# Autodesk Inventor assembly: Rover_komplett
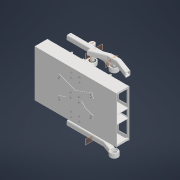
[picture p0: Inventor's stored thumbnail of the model, 180x180]
Saved by Autodesk Inventor 2021 (Build 250183000, 183)
## iProperties
Created: 2021-03-06
Part Number: Rover_komplett
Document SubType Name: Assembly
Designer: Ctroi
Author: Ctroi
## Documents named in this file (25)
- G:\Roverprojekt\Github Projekt\Rover\Rover_komplett.iam
- G:\Roverprojekt\Github Projekt\Rover\Grundplatte_vorne.ipt
- G:\Roverprojekt\Github Projekt\Rover\Grundplatte_hinten.ipt
- G:\Roverprojekt\Github Projekt\Rover\Obenplatte_vorne.ipt
- C:\Users\Ctroi\Documents\Inventor\Content Center Files\R2021\de-DE\ISO 7089\ISO 7089 - 3 - 140 HV(1).ipt
- C:\Users\Ctroi\Documents\Inventor\Content Center Files\R2021\de-DE\BS 4168(1)\BS 4168 - M3 x 10(1).ipt
- C:\Users\Ctroi\Documents\Inventor\Content Center Files\R2021\de-DE\ANSI B18.16.3M(2)\ANSI B18.16.3M - Property Class 5 and 10 - Metric M3 x 0.5 Metallisch.ipt
- G:\Roverprojekt\Github Projekt\Rover\Kreuz_Halterung.ipt
- C:\Users\Ctroi\Documents\Inventor\Content Center Files\R2021\de-DE\BS 4168(1)\BS 4168 - M3 x 8(1).ipt
- G:\Roverprojekt\Github Projekt\Rover\Obenplatte_hinten.ipt
- G:\Roverprojekt\Github Projekt\Rover\Halterung_Differential_3.ipt
- C:\Users\Ctroi\Documents\Inventor\Content Center Files\R2021\de-DE\BS 4168(1)\BS 4168 - M3 x 12(1).ipt
- G:\Roverprojekt\Github Projekt\Rover\Halterung_Differential.ipt
- G:\Roverprojekt\Github Projekt\Rover\Halterung_Differential_2.ipt
- G:\Roverprojekt\Github Projekt\Rover\Kugellager.ipt
- G:\Roverprojekt\Github Projekt\Rover\Halterung_Differential_Mitte.ipt
- G:\Roverprojekt\Github Projekt\Rover\Kugellager_klein.ipt
- G:\Roverprojekt\Github Projekt\Rover\Welle_Kugellager_Mitte.ipt
- G:\Roverprojekt\Github Projekt\Rover\Kegelrad.ipt
- G:\Roverprojekt\Github Projekt\Rover\Verbindung_Rocker_Body.ipt
- C:\Users\Ctroi\Documents\Inventor\Content Center Files\R2021\de-DE\BS 4168(1)\BS 4168 - M3 x 16(1).ipt
- G:\Roverprojekt\Github Projekt\Rover\Rocker_hinten.ipt
- G:\Roverprojekt\Github Projekt\Rover\Rocker_hinten_rechts.ipt
- G:\Roverprojekt\Github Projekt\Rover\Boogie_Stange.ipt
- G:\Roverprojekt\Github Projekt\Rover\Bogie.ipt
## Components (165 placed, 23 different names)
1. Fahrwerk_rocker_hinten:1 — Passend:196, Passend:197, Winkel:8, Passend:200, Passend:201, Passend:202, Passend:203
2. Fahrwerk_rocker_hinten:2 — Passend:198, Passend:199, Winkel:9
3. Kugellager:6 — Passend:200, Passend:201, Einfügen:72
4. Kugellager:7 — Passend:202, Passend:203
5. Boogie_Stange:1 — Einfügen:72, Passend:204, Passend:205, Winkel:10
6. Fahrwerk_bogie:1 — Passend:204, Passend:205, Winkel:10
7. ISO 7089 3:17 — Passend:46, Passend:47, Einfügen:17
8. BS 4168 : Teil 1 Innensechskantschraube - Metrisch M3 x 8:1 — Einfügen:17
9. ISO 7089 3:18 — Passend:48, Passend:49, Einfügen:18
10. Sechskantmutter mit Sicherungselement - Stahl Metrisch Property Class 5 and 10 - Metric M3 x 0.5 Metallisch:9 — Einfügen:18
11. ISO 7089 3:19 — Passend:50, Passend:51, Einfügen:19
12. BS 4168 : Teil 1 Innensechskantschraube - Metrisch M3 x 8:2 — Einfügen:19
13. ISO 7089 3:20 — Passend:52, Passend:53, Einfügen:20
14. Sechskantmutter mit Sicherungselement - Stahl Metrisch Property Class 5 and 10 - Metric M3 x 0.5 Metallisch:10 — Einfügen:20
15. ISO 7089 3:21 — Passend:54, Passend:55, Einfügen:21
16. BS 4168 : Teil 1 Innensechskantschraube - Metrisch M3 x 8:3 — Einfügen:21
17. ISO 7089 3:22 — Passend:56, Passend:57, Einfügen:22
18. Sechskantmutter mit Sicherungselement - Stahl Metrisch Property Class 5 and 10 - Metric M3 x 0.5 Metallisch:11 — Einfügen:22
19. ISO 7089 3:23 — Passend:58, Passend:59, Einfügen:23
20. BS 4168 : Teil 1 Innensechskantschraube - Metrisch M3 x 8:4 — Einfügen:23
21. ISO 7089 3:24 — Passend:60, Passend:61, Einfügen:24
22. Sechskantmutter mit Sicherungselement - Stahl Metrisch Property Class 5 and 10 - Metric M3 x 0.5 Metallisch:12 — Einfügen:24
23. ISO 7089 3:25 — Passend:62, Passend:63, Einfügen:25
24. BS 4168 : Teil 1 Innensechskantschraube - Metrisch M3 x 8:5 — Einfügen:25
25. ISO 7089 3:26 — Passend:64, Passend:65, Einfügen:26
26. Sechskantmutter mit Sicherungselement - Stahl Metrisch Property Class 5 and 10 - Metric M3 x 0.5 Metallisch:13 — Einfügen:26
27. ISO 7089 3:27 — Passend:66, Passend:67, Einfügen:27
28. BS 4168 : Teil 1 Innensechskantschraube - Metrisch M3 x 10:9 — Einfügen:27
29. ISO 7089 3:28 — Passend:68, Passend:69, Einfügen:28
30. Sechskantmutter mit Sicherungselement - Stahl Metrisch Property Class 5 and 10 - Metric M3 x 0.5 Metallisch:14 — Einfügen:28
31. ISO 7089 3:29 — Passend:70, Passend:71, Einfügen:29
32. BS 4168 : Teil 1 Innensechskantschraube - Metrisch M3 x 10:10 — Einfügen:29
33. ISO 7089 3:30 — Passend:72, Passend:73, Einfügen:30
34. Sechskantmutter mit Sicherungselement - Stahl Metrisch Property Class 5 and 10 - Metric M3 x 0.5 Metallisch:15 — Einfügen:30
35. ISO 7089 3:31 — Passend:74, Passend:75, Einfügen:31
36. BS 4168 : Teil 1 Innensechskantschraube - Metrisch M3 x 10:11 — Einfügen:31
37. ISO 7089 3:32 — Passend:76, Passend:77, Einfügen:32
38. Sechskantmutter mit Sicherungselement - Stahl Metrisch Property Class 5 and 10 - Metric M3 x 0.5 Metallisch:16 — Einfügen:32
39. ISO 7089 3:33 — Passend:78, Passend:79, Einfügen:33
40. BS 4168 : Teil 1 Innensechskantschraube - Metrisch M3 x 10:12 — Einfügen:33
41. ISO 7089 3:34 — Passend:80, Passend:81, Einfügen:34
42. Sechskantmutter mit Sicherungselement - Stahl Metrisch Property Class 5 and 10 - Metric M3 x 0.5 Metallisch:17 — Einfügen:34
43. ISO 7089 3:35 — Passend:82, Passend:83, Einfügen:35
44. BS 4168 : Teil 1 Innensechskantschraube - Metrisch M3 x 10:13 — Einfügen:35
45. ISO 7089 3:36 — Passend:84, Passend:85, Einfügen:36
46. Sechskantmutter mit Sicherungselement - Stahl Metrisch Property Class 5 and 10 - Metric M3 x 0.5 Metallisch:18 — Einfügen:36
47. ISO 7089 3:37 — Passend:86, Passend:87, Einfügen:37
48. BS 4168 : Teil 1 Innensechskantschraube - Metrisch M3 x 10:14 — Einfügen:37
49. ISO 7089 3:38 — Passend:88, Passend:89, Einfügen:38
50. Sechskantmutter mit Sicherungselement - Stahl Metrisch Property Class 5 and 10 - Metric M3 x 0.5 Metallisch:19 — Einfügen:38
51. ISO 7089 3:39 — Passend:90, Passend:91, Einfügen:39
52. BS 4168 : Teil 1 Innensechskantschraube - Metrisch M3 x 10:15 — Einfügen:39
53. ISO 7089 3:40 — Passend:92, Passend:93, Einfügen:40
54. Sechskantmutter mit Sicherungselement - Stahl Metrisch Property Class 5 and 10 - Metric M3 x 0.5 Metallisch:20 — Einfügen:40
55. ISO 7089 3:1 — Passend:11, Passend:12, Einfügen:1
56. BS 4168 : Teil 1 Innensechskantschraube - Metrisch M3 x 10:1 — Einfügen:1
57. ISO 7089 3:2 — Passend:13, Passend:14, Einfügen:2
58. Sechskantmutter mit Sicherungselement - Stahl Metrisch Property Class 5 and 10 - Metric M3 x 0.5 Metallisch:1 — Einfügen:2
59. ISO 7089 3:3 — Passend:15, Passend:16, Einfügen:3
60. BS 4168 : Teil 1 Innensechskantschraube - Metrisch M3 x 10:2 — Einfügen:3
61. ISO 7089 3:4 — Passend:17, Passend:18, Einfügen:4
62. Sechskantmutter mit Sicherungselement - Stahl Metrisch Property Class 5 and 10 - Metric M3 x 0.5 Metallisch:2 — Einfügen:4
63. ISO 7089 3:5 — Passend:19, Passend:20, Einfügen:5
64. BS 4168 : Teil 1 Innensechskantschraube - Metrisch M3 x 10:3 — Einfügen:5
65. ISO 7089 3:6 — Passend:21, Passend:22, Einfügen:6
66. Sechskantmutter mit Sicherungselement - Stahl Metrisch Property Class 5 and 10 - Metric M3 x 0.5 Metallisch:3 — Einfügen:6
67. ISO 7089 3:7 — Passend:23, Passend:24, Einfügen:7
68. BS 4168 : Teil 1 Innensechskantschraube - Metrisch M3 x 10:4 — Einfügen:7
69. ISO 7089 3:8 — Passend:25, Passend:26, Einfügen:8
70. Sechskantmutter mit Sicherungselement - Stahl Metrisch Property Class 5 and 10 - Metric M3 x 0.5 Metallisch:4 — Einfügen:8
71. ISO 7089 3:9 — Passend:27, Passend:28, Einfügen:9
72. BS 4168 : Teil 1 Innensechskantschraube - Metrisch M3 x 10:5 — Einfügen:9
73. ISO 7089 3:10 — Passend:29, Passend:30, Einfügen:10
74. Sechskantmutter mit Sicherungselement - Stahl Metrisch Property Class 5 and 10 - Metric M3 x 0.5 Metallisch:5 — Einfügen:10
75. ISO 7089 3:11 — Passend:31, Passend:32, Einfügen:11
76. BS 4168 : Teil 1 Innensechskantschraube - Metrisch M3 x 10:6 — Einfügen:11
77. ISO 7089 3:12 — Passend:33, Passend:34, Einfügen:12
78. Sechskantmutter mit Sicherungselement - Stahl Metrisch Property Class 5 and 10 - Metric M3 x 0.5 Metallisch:6 — Einfügen:12
79. ISO 7089 3:13 — Passend:35, Passend:36, Einfügen:13
80. BS 4168 : Teil 1 Innensechskantschraube - Metrisch M3 x 10:7 — Einfügen:13
81. ISO 7089 3:14 — Passend:37, Passend:38, Einfügen:14
82. Sechskantmutter mit Sicherungselement - Stahl Metrisch Property Class 5 and 10 - Metric M3 x 0.5 Metallisch:7 — Einfügen:14
83. ISO 7089 3:15 — Passend:39, Passend:40, Einfügen:15
84. BS 4168 : Teil 1 Innensechskantschraube - Metrisch M3 x 10:8 — Einfügen:15
85. ISO 7089 3:16 — Passend:41, Passend:42, Einfügen:16
86. Sechskantmutter mit Sicherungselement - Stahl Metrisch Property Class 5 and 10 - Metric M3 x 0.5 Metallisch:8 — Einfügen:16
87. ISO 7089 3:57 — Passend:172, Passend:173, Einfügen:60
88. BS 4168 : Teil 1 Innensechskantschraube - Metrisch M3 x 12:5 — Einfügen:60
89. ISO 7089 3:58 — Passend:174, Passend:175, Einfügen:61
90. Sechskantmutter mit Sicherungselement - Stahl Metrisch Property Class 5 and 10 - Metric M3 x 0.5 Metallisch:25 — Einfügen:61
91. ISO 7089 3:59 — Passend:176, Passend:177, Einfügen:62
92. BS 4168 : Teil 1 Innensechskantschraube - Metrisch M3 x 12:6 — Einfügen:62
93. ISO 7089 3:60 — Passend:178, Passend:179, Einfügen:63
94. Sechskantmutter mit Sicherungselement - Stahl Metrisch Property Class 5 and 10 - Metric M3 x 0.5 Metallisch:26 — Einfügen:63
95. ISO 7089 3:61 — Passend:180, Passend:181, Einfügen:64
96. BS 4168 : Teil 1 Innensechskantschraube - Metrisch M3 x 16:1 — Einfügen:64
97. ISO 7089 3:62 — Passend:182, Passend:183, Einfügen:65
98. Sechskantmutter mit Sicherungselement - Stahl Metrisch Property Class 5 and 10 - Metric M3 x 0.5 Metallisch:27 — Einfügen:65
99. ISO 7089 3:63 — Passend:184, Passend:185, Einfügen:66
100. BS 4168 : Teil 1 Innensechskantschraube - Metrisch M3 x 12:7 — Einfügen:66
101. ISO 7089 3:64 — Passend:186, Passend:187, Einfügen:67
102. Sechskantmutter mit Sicherungselement - Stahl Metrisch Property Class 5 and 10 - Metric M3 x 0.5 Metallisch:28 — Einfügen:67
103. ISO 7089 3:65 — Passend:188, Passend:189, Einfügen:68
104. BS 4168 : Teil 1 Innensechskantschraube - Metrisch M3 x 12:8 — Einfügen:68
105. ISO 7089 3:66 — Passend:190, Passend:191, Einfügen:69
106. Sechskantmutter mit Sicherungselement - Stahl Metrisch Property Class 5 and 10 - Metric M3 x 0.5 Metallisch:29 — Einfügen:69
107. ISO 7089 3:67 — Passend:192, Passend:193, Einfügen:70
108. BS 4168 : Teil 1 Innensechskantschraube - Metrisch M3 x 16:2 — Einfügen:70
109. ISO 7089 3:68 — Passend:194, Passend:195, Einfügen:71
110. Sechskantmutter mit Sicherungselement - Stahl Metrisch Property Class 5 and 10 - Metric M3 x 0.5 Metallisch:30 — Einfügen:71
111. ISO 7089 3:49 — Passend:119, Passend:120, Einfügen:49
112. BS 4168 : Teil 1 Innensechskantschraube - Metrisch M3 x 12:1 — Einfügen:49
113. ISO 7089 3:50 — Passend:121, Passend:122, Einfügen:50
114. Sechskantmutter mit Sicherungselement - Stahl Metrisch Property Class 5 and 10 - Metric M3 x 0.5 Metallisch:21 — Einfügen:50
115. ISO 7089 3:51 — Passend:123, Passend:124, Einfügen:51
116. BS 4168 : Teil 1 Innensechskantschraube - Metrisch M3 x 12:2 — Einfügen:51
117. ISO 7089 3:52 — Passend:125, Passend:126, Einfügen:52
118. Sechskantmutter mit Sicherungselement - Stahl Metrisch Property Class 5 and 10 - Metric M3 x 0.5 Metallisch:22 — Einfügen:52
119. ISO 7089 3:53 — Passend:127, Passend:128, Einfügen:53
120. BS 4168 : Teil 1 Innensechskantschraube - Metrisch M3 x 12:3 — Einfügen:53
121. ISO 7089 3:54 — Passend:129, Passend:130, Einfügen:54
122. Sechskantmutter mit Sicherungselement - Stahl Metrisch Property Class 5 and 10 - Metric M3 x 0.5 Metallisch:23 — Einfügen:54
123. ISO 7089 3:55 — Passend:131, Passend:132, Einfügen:55
124. BS 4168 : Teil 1 Innensechskantschraube - Metrisch M3 x 12:4 — Einfügen:55
125. ISO 7089 3:56 — Passend:133, Passend:134, Einfügen:56
126. Sechskantmutter mit Sicherungselement - Stahl Metrisch Property Class 5 and 10 - Metric M3 x 0.5 Metallisch:24 — Einfügen:56
127. ISO 7089 3:42 — Passend:96, Passend:97, Einfügen:42
128. BS 4168 : Teil 1 Innensechskantschraube - Metrisch M3 x 8:7 — Einfügen:42
129. ISO 7089 3:43 — Passend:98, Passend:99, Einfügen:43
130. BS 4168 : Teil 1 Innensechskantschraube - Metrisch M3 x 8:8 — Einfügen:43
131. ISO 7089 3:44 — Passend:100, Passend:101, Einfügen:44
132. BS 4168 : Teil 1 Innensechskantschraube - Metrisch M3 x 8:9 — Einfügen:44
133. ISO 7089 3:45 — Passend:105, Passend:106, Einfügen:45
134. BS 4168 : Teil 1 Innensechskantschraube - Metrisch M3 x 8:10 — Einfügen:45
135. ISO 7089 3:46 — Passend:107, Passend:108, Einfügen:46
136. BS 4168 : Teil 1 Innensechskantschraube - Metrisch M3 x 8:11 — Einfügen:46
137. ISO 7089 3:47 — Passend:109, Passend:110, Einfügen:47
138. BS 4168 : Teil 1 Innensechskantschraube - Metrisch M3 x 8:12 — Einfügen:47
139. ISO 7089 3:48 — Passend:111, Passend:112, Einfügen:48
140. BS 4168 : Teil 1 Innensechskantschraube - Metrisch M3 x 8:13 — Einfügen:48
141. ISO 7089 3:41 — Passend:94, Passend:95, Einfügen:41
142. BS 4168 : Teil 1 Innensechskantschraube - Metrisch M3 x 8:6 — Einfügen:41
143. Kegelrad2:3 — Passend:170, Passend:171, Winkel:7, Drehung:2
144. Kegelrad2:2 — Passend:168, Passend:169, Winkel:4, Drehung:1
145. Verbindung_Rocker_Body:2 — Einfügen:58, Passend:168, Passend:169, Winkel:4, Passend:196, Passend:197, Winkel:8
146. Verbindung_Rocker_Body:1 — Einfügen:59, Passend:170, Passend:171, Winkel:7, Passend:198, Passend:199, Winkel:9
147. Kegelrad2:1 — Passend:166, Passend:167, Drehung:1, Winkel:5, Winkel:6, Drehung:2
148. Halterung_Differential:1 — Passend:140, Passend:146, Passend:147, Passend:148, Passend:157, Passend:158, Passend:176, Passend:177, Passend:178
149. Halterung_Differential:2 — Passend:137, Passend:144, Passend:145, Passend:149, Passend:155, Passend:156, Passend:172, Passend:173, Passend:174
150. Halterung_Differential_2:1 — Passend:148, Passend:149, Passend:152, Passend:153, Passend:154, Passend:180, Passend:181, Passend:182, Passend:192, Passend:193, Passend:194
151. Kugellager:1 — Passend:152, Passend:154
152. Kugellager:2 — Passend:155, Passend:156
153. Kugellager:3 — Passend:150, Passend:151, Einfügen:59
154. Kugellager:4 — Passend:157, Passend:158
155. Kugellager:5 — Passend:159, Passend:160, Einfügen:58
156. Halterung_Differential_Mitte:1 — Passend:161, Passend:162, Passend:163, Passend:164, Passend:165, Passend:184, Passend:185, Passend:186, Passend:188, Passend:189, Passend:190
157. Kugellager_klein:1 — Passend:164, Passend:165, Einfügen:57
158. Welle_Kugellager_Mitte:1 — Einfügen:57, Passend:166, Passend:167, Winkel:5
159. Obenplatte_hinten:1 — Passend:102, Passend:103, Passend:104, Passend:105, Passend:106, Passend:107, Passend:108, Passend:109, Passend:110, Passend:111, Passend:112, Passend:114, Passend:115, Passend:117, Passend:118, Passend:122, Passend:130, Passend:140, Passend:145, Passend:146, Passend:175, Passend:179
160. Obenplatte_vorne:1 — Passend:4, Passend:5, Passend:6, Passend:94, Passend:95, Passend:96, Passend:97, Passend:98, Passend:99, Passend:100, Passend:101, Passend:113, Passend:116, Passend:126, Passend:134, Passend:137, Passend:144, Passend:147, Passend:153, Passend:161, Passend:162, Passend:163, Winkel:6, Passend:183, Passend:187, Passend:191, Passend:195
161. Halterung_Differential_3:1 — Passend:113, Passend:114, Passend:115, Passend:127, Passend:128, Passend:129, Passend:131, Passend:132, Passend:133, Passend:159, Passend:160
162. Halterung_Differential_3:2 — Passend:116, Passend:117, Passend:118, Passend:119, Passend:120, Passend:121, Passend:123, Passend:124, Passend:125, Passend:150, Passend:151
163. Grundplatte_vorne:1 — Passend:1, Passend:2, Passend:3, Passend:4, Passend:5, Passend:6, Passend:22, Passend:26, Passend:30, Passend:34, Passend:43, Passend:46, Passend:47, Passend:48, Passend:49, Passend:50, Passend:51, Passend:52, Passend:53, Passend:54, Passend:55, Passend:56, Passend:57, Passend:58, Passend:59, Passend:60, Passend:61, Passend:78, Passend:79, Passend:80, Passend:82, Passend:83, Passend:84
164. Grundplatte_hinten:1 — Passend:1, Passend:2, Passend:3, Passend:11, Passend:12, Passend:13, Passend:14, Passend:15, Passend:16, Passend:17, Passend:18, Passend:19, Passend:20, Passend:21, Passend:23, Passend:24, Passend:25, Passend:27, Passend:28, Passend:29, Passend:31, Passend:32, Passend:33, Passend:35, Passend:36, Passend:37, Passend:38, Passend:39, Passend:40, Passend:41, Passend:42, Passend:44, Passend:45, Passend:62, Passend:63, Passend:64, Passend:65, Passend:66, Passend:67, Passend:68, Passend:70, Passend:71, Passend:72, Passend:74, Passend:75, Passend:76, Passend:86, Passend:87, Passend:88, Passend:90, Passend:91, Passend:92, Passend:102, Passend:103, Passend:104
165. Kreuz_Halterung:1 — Passend:43, Passend:44, Passend:45, Passend:69, Passend:73, Passend:77, Passend:81, Passend:85, Passend:89, Passend:93
## Relationships (275: Mate 194, Insert 72, Angle 7, RelateRotation 2)
- Passend:1 [Mate]: Grundplatte_vorne:1 ↔ Grundplatte_hinten:1
- Passend:2 [Mate]: Grundplatte_vorne:1 ↔ Grundplatte_hinten:1
- Passend:3 [Mate]: Grundplatte_vorne:1 ↔ Grundplatte_hinten:1
- Passend:4 [Mate]: Obenplatte_vorne:1 ↔ Grundplatte_vorne:1
- Passend:5 [Mate]: Obenplatte_vorne:1 ↔ Grundplatte_vorne:1
- Passend:6 [Mate]: Obenplatte_vorne:1 ↔ Grundplatte_vorne:1
- Passend:11 [Mate]: ISO 7089 3:1 ↔ Grundplatte_hinten:1
- Passend:12 [Mate]: ISO 7089 3:1 ↔ Grundplatte_hinten:1
- Einfügen:1 [Insert]: ISO 7089 3:1 ↔ BS 4168 : Teil 1 Innensechskantschraube - Metrisch M3 x 10:1
- Passend:13 [Mate]: ISO 7089 3:2 ↔ Grundplatte_hinten:1
- Passend:14 [Mate]: ISO 7089 3:2 ↔ Grundplatte_hinten:1
- Einfügen:2 [Insert]: ISO 7089 3:2 ↔ Sechskantmutter mit Sicherungselement - Stahl Metrisch Property Class 5 and 10 - Metric M3 x 0.5 Metallisch:1
- Passend:15 [Mate]: ISO 7089 3:3 ↔ Grundplatte_hinten:1
- Passend:16 [Mate]: ISO 7089 3:3 ↔ Grundplatte_hinten:1
- Einfügen:3 [Insert]: ISO 7089 3:3 ↔ BS 4168 : Teil 1 Innensechskantschraube - Metrisch M3 x 10:2
- Passend:17 [Mate]: ISO 7089 3:4 ↔ Grundplatte_hinten:1
- Passend:18 [Mate]: ISO 7089 3:4 ↔ Grundplatte_hinten:1
- Einfügen:4 [Insert]: ISO 7089 3:4 ↔ Sechskantmutter mit Sicherungselement - Stahl Metrisch Property Class 5 and 10 - Metric M3 x 0.5 Metallisch:2
- Passend:19 [Mate]: ISO 7089 3:5 ↔ Grundplatte_hinten:1
- Passend:20 [Mate]: ISO 7089 3:5 ↔ Grundplatte_hinten:1
- Einfügen:5 [Insert]: ISO 7089 3:5 ↔ BS 4168 : Teil 1 Innensechskantschraube - Metrisch M3 x 10:3
- Passend:21 [Mate]: ISO 7089 3:6 ↔ Grundplatte_hinten:1
- Passend:22 [Mate]: ISO 7089 3:6 ↔ Grundplatte_vorne:1
- Einfügen:6 [Insert]: ISO 7089 3:6 ↔ Sechskantmutter mit Sicherungselement - Stahl Metrisch Property Class 5 and 10 - Metric M3 x 0.5 Metallisch:3
- Passend:23 [Mate]: ISO 7089 3:7 ↔ Grundplatte_hinten:1
- Passend:24 [Mate]: ISO 7089 3:7 ↔ Grundplatte_hinten:1
- Einfügen:7 [Insert]: ISO 7089 3:7 ↔ BS 4168 : Teil 1 Innensechskantschraube - Metrisch M3 x 10:4
- Passend:25 [Mate]: ISO 7089 3:8 ↔ Grundplatte_hinten:1
- Passend:26 [Mate]: ISO 7089 3:8 ↔ Grundplatte_vorne:1
- Einfügen:8 [Insert]: ISO 7089 3:8 ↔ Sechskantmutter mit Sicherungselement - Stahl Metrisch Property Class 5 and 10 - Metric M3 x 0.5 Metallisch:4
- Passend:27 [Mate]: ISO 7089 3:9 ↔ Grundplatte_hinten:1
- Passend:28 [Mate]: ISO 7089 3:9 ↔ Grundplatte_hinten:1
- Einfügen:9 [Insert]: ISO 7089 3:9 ↔ BS 4168 : Teil 1 Innensechskantschraube - Metrisch M3 x 10:5
- Passend:29 [Mate]: ISO 7089 3:10 ↔ Grundplatte_hinten:1
- Passend:30 [Mate]: ISO 7089 3:10 ↔ Grundplatte_vorne:1
- Einfügen:10 [Insert]: ISO 7089 3:10 ↔ Sechskantmutter mit Sicherungselement - Stahl Metrisch Property Class 5 and 10 - Metric M3 x 0.5 Metallisch:5
- Passend:31 [Mate]: ISO 7089 3:11 ↔ Grundplatte_hinten:1
- Passend:32 [Mate]: ISO 7089 3:11 ↔ Grundplatte_hinten:1
- Einfügen:11 [Insert]: ISO 7089 3:11 ↔ BS 4168 : Teil 1 Innensechskantschraube - Metrisch M3 x 10:6
- Passend:33 [Mate]: ISO 7089 3:12 ↔ Grundplatte_hinten:1
- Passend:34 [Mate]: ISO 7089 3:12 ↔ Grundplatte_vorne:1
- Einfügen:12 [Insert]: ISO 7089 3:12 ↔ Sechskantmutter mit Sicherungselement - Stahl Metrisch Property Class 5 and 10 - Metric M3 x 0.5 Metallisch:6
- Passend:35 [Mate]: ISO 7089 3:13 ↔ Grundplatte_hinten:1
- Passend:36 [Mate]: ISO 7089 3:13 ↔ Grundplatte_hinten:1
- Einfügen:13 [Insert]: ISO 7089 3:13 ↔ BS 4168 : Teil 1 Innensechskantschraube - Metrisch M3 x 10:7
- Passend:37 [Mate]: ISO 7089 3:14 ↔ Grundplatte_hinten:1
- Passend:38 [Mate]: ISO 7089 3:14 ↔ Grundplatte_hinten:1
- Einfügen:14 [Insert]: ISO 7089 3:14 ↔ Sechskantmutter mit Sicherungselement - Stahl Metrisch Property Class 5 and 10 - Metric M3 x 0.5 Metallisch:7
- Passend:39 [Mate]: ISO 7089 3:15 ↔ Grundplatte_hinten:1
- Passend:40 [Mate]: ISO 7089 3:15 ↔ Grundplatte_hinten:1
- Einfügen:15 [Insert]: ISO 7089 3:15 ↔ BS 4168 : Teil 1 Innensechskantschraube - Metrisch M3 x 10:8
- Passend:41 [Mate]: ISO 7089 3:16 ↔ Grundplatte_hinten:1
- Passend:42 [Mate]: ISO 7089 3:16 ↔ Grundplatte_hinten:1
- Einfügen:16 [Insert]: ISO 7089 3:16 ↔ Sechskantmutter mit Sicherungselement - Stahl Metrisch Property Class 5 and 10 - Metric M3 x 0.5 Metallisch:8
- Passend:43 [Mate]: Grundplatte_vorne:1 ↔ Kreuz_Halterung:1
- Passend:44 [Mate]: Grundplatte_hinten:1 ↔ Kreuz_Halterung:1
- Passend:45 [Mate]: Grundplatte_hinten:1 ↔ Kreuz_Halterung:1
- Passend:46 [Mate]: ISO 7089 3:17 ↔ Grundplatte_vorne:1
- Passend:47 [Mate]: ISO 7089 3:17 ↔ Grundplatte_vorne:1
- Einfügen:17 [Insert]: ISO 7089 3:17 ↔ BS 4168 : Teil 1 Innensechskantschraube - Metrisch M3 x 8:1
- Passend:48 [Mate]: ISO 7089 3:18 ↔ Grundplatte_vorne:1
- Passend:49 [Mate]: ISO 7089 3:18 ↔ Grundplatte_vorne:1
- Einfügen:18 [Insert]: ISO 7089 3:18 ↔ Sechskantmutter mit Sicherungselement - Stahl Metrisch Property Class 5 and 10 - Metric M3 x 0.5 Metallisch:9
- Passend:50 [Mate]: ISO 7089 3:19 ↔ Grundplatte_vorne:1
- Passend:51 [Mate]: ISO 7089 3:19 ↔ Grundplatte_vorne:1
- Einfügen:19 [Insert]: ISO 7089 3:19 ↔ BS 4168 : Teil 1 Innensechskantschraube - Metrisch M3 x 8:2
- Passend:52 [Mate]: ISO 7089 3:20 ↔ Grundplatte_vorne:1
- Passend:53 [Mate]: ISO 7089 3:20 ↔ Grundplatte_vorne:1
- Einfügen:20 [Insert]: ISO 7089 3:20 ↔ Sechskantmutter mit Sicherungselement - Stahl Metrisch Property Class 5 and 10 - Metric M3 x 0.5 Metallisch:10
- Passend:54 [Mate]: ISO 7089 3:21 ↔ Grundplatte_vorne:1
- Passend:55 [Mate]: ISO 7089 3:21 ↔ Grundplatte_vorne:1
- Einfügen:21 [Insert]: ISO 7089 3:21 ↔ BS 4168 : Teil 1 Innensechskantschraube - Metrisch M3 x 8:3
- Passend:56 [Mate]: ISO 7089 3:22 ↔ Grundplatte_vorne:1
- Passend:57 [Mate]: ISO 7089 3:22 ↔ Grundplatte_vorne:1
- Einfügen:22 [Insert]: ISO 7089 3:22 ↔ Sechskantmutter mit Sicherungselement - Stahl Metrisch Property Class 5 and 10 - Metric M3 x 0.5 Metallisch:11
- Passend:58 [Mate]: ISO 7089 3:23 ↔ Grundplatte_vorne:1
- Passend:59 [Mate]: ISO 7089 3:23 ↔ Grundplatte_vorne:1
- Einfügen:23 [Insert]: ISO 7089 3:23 ↔ BS 4168 : Teil 1 Innensechskantschraube - Metrisch M3 x 8:4
- Passend:60 [Mate]: ISO 7089 3:24 ↔ Grundplatte_vorne:1
- Passend:61 [Mate]: ISO 7089 3:24 ↔ Grundplatte_vorne:1
- Einfügen:24 [Insert]: ISO 7089 3:24 ↔ Sechskantmutter mit Sicherungselement - Stahl Metrisch Property Class 5 and 10 - Metric M3 x 0.5 Metallisch:12
- Passend:62 [Mate]: ISO 7089 3:25 ↔ Grundplatte_hinten:1
- Passend:63 [Mate]: ISO 7089 3:25 ↔ Grundplatte_hinten:1
- Einfügen:25 [Insert]: ISO 7089 3:25 ↔ BS 4168 : Teil 1 Innensechskantschraube - Metrisch M3 x 8:5
- Passend:64 [Mate]: ISO 7089 3:26 ↔ Grundplatte_hinten:1
- Passend:65 [Mate]: ISO 7089 3:26 ↔ Grundplatte_hinten:1
- Einfügen:26 [Insert]: ISO 7089 3:26 ↔ Sechskantmutter mit Sicherungselement - Stahl Metrisch Property Class 5 and 10 - Metric M3 x 0.5 Metallisch:13
- Passend:66 [Mate]: ISO 7089 3:27 ↔ Grundplatte_hinten:1
- Passend:67 [Mate]: ISO 7089 3:27 ↔ Grundplatte_hinten:1
- Einfügen:27 [Insert]: ISO 7089 3:27 ↔ BS 4168 : Teil 1 Innensechskantschraube - Metrisch M3 x 10:9
- Passend:68 [Mate]: ISO 7089 3:28 ↔ Grundplatte_hinten:1
- Passend:69 [Mate]: ISO 7089 3:28 ↔ Kreuz_Halterung:1
- Einfügen:28 [Insert]: ISO 7089 3:28 ↔ Sechskantmutter mit Sicherungselement - Stahl Metrisch Property Class 5 and 10 - Metric M3 x 0.5 Metallisch:14
- Passend:70 [Mate]: ISO 7089 3:29 ↔ Grundplatte_hinten:1
- Passend:71 [Mate]: ISO 7089 3:29 ↔ Grundplatte_hinten:1
- Einfügen:29 [Insert]: ISO 7089 3:29 ↔ BS 4168 : Teil 1 Innensechskantschraube - Metrisch M3 x 10:10
- Passend:72 [Mate]: ISO 7089 3:30 ↔ Grundplatte_hinten:1
- Passend:73 [Mate]: ISO 7089 3:30 ↔ Kreuz_Halterung:1
- Einfügen:30 [Insert]: ISO 7089 3:30 ↔ Sechskantmutter mit Sicherungselement - Stahl Metrisch Property Class 5 and 10 - Metric M3 x 0.5 Metallisch:15
- Passend:74 [Mate]: ISO 7089 3:31 ↔ Grundplatte_hinten:1
- Passend:75 [Mate]: ISO 7089 3:31 ↔ Grundplatte_hinten:1
- Einfügen:31 [Insert]: ISO 7089 3:31 ↔ BS 4168 : Teil 1 Innensechskantschraube - Metrisch M3 x 10:11
- Passend:76 [Mate]: ISO 7089 3:32 ↔ Grundplatte_hinten:1
- Passend:77 [Mate]: ISO 7089 3:32 ↔ Kreuz_Halterung:1
- Einfügen:32 [Insert]: ISO 7089 3:32 ↔ Sechskantmutter mit Sicherungselement - Stahl Metrisch Property Class 5 and 10 - Metric M3 x 0.5 Metallisch:16
- Passend:78 [Mate]: ISO 7089 3:33 ↔ Grundplatte_vorne:1
- Passend:79 [Mate]: ISO 7089 3:33 ↔ Grundplatte_vorne:1
- Einfügen:33 [Insert]: ISO 7089 3:33 ↔ BS 4168 : Teil 1 Innensechskantschraube - Metrisch M3 x 10:12
- Passend:80 [Mate]: ISO 7089 3:34 ↔ Grundplatte_vorne:1
- Passend:81 [Mate]: ISO 7089 3:34 ↔ Kreuz_Halterung:1
- Einfügen:34 [Insert]: ISO 7089 3:34 ↔ Sechskantmutter mit Sicherungselement - Stahl Metrisch Property Class 5 and 10 - Metric M3 x 0.5 Metallisch:17
- Passend:82 [Mate]: ISO 7089 3:35 ↔ Grundplatte_vorne:1
- Passend:83 [Mate]: ISO 7089 3:35 ↔ Grundplatte_vorne:1
- Einfügen:35 [Insert]: ISO 7089 3:35 ↔ BS 4168 : Teil 1 Innensechskantschraube - Metrisch M3 x 10:13
- Passend:84 [Mate]: ISO 7089 3:36 ↔ Grundplatte_vorne:1
- Passend:85 [Mate]: ISO 7089 3:36 ↔ Kreuz_Halterung:1
- Einfügen:36 [Insert]: ISO 7089 3:36 ↔ Sechskantmutter mit Sicherungselement - Stahl Metrisch Property Class 5 and 10 - Metric M3 x 0.5 Metallisch:18
- Passend:86 [Mate]: ISO 7089 3:37 ↔ Grundplatte_hinten:1
- Passend:87 [Mate]: ISO 7089 3:37 ↔ Grundplatte_hinten:1
- Einfügen:37 [Insert]: ISO 7089 3:37 ↔ BS 4168 : Teil 1 Innensechskantschraube - Metrisch M3 x 10:14
- Passend:88 [Mate]: ISO 7089 3:38 ↔ Grundplatte_hinten:1
- Passend:89 [Mate]: ISO 7089 3:38 ↔ Kreuz_Halterung:1
- Einfügen:38 [Insert]: ISO 7089 3:38 ↔ Sechskantmutter mit Sicherungselement - Stahl Metrisch Property Class 5 and 10 - Metric M3 x 0.5 Metallisch:19
- Passend:90 [Mate]: ISO 7089 3:39 ↔ Grundplatte_hinten:1
- Passend:91 [Mate]: ISO 7089 3:39 ↔ Grundplatte_hinten:1
- Einfügen:39 [Insert]: ISO 7089 3:39 ↔ BS 4168 : Teil 1 Innensechskantschraube - Metrisch M3 x 10:15
- Passend:92 [Mate]: ISO 7089 3:40 ↔ Grundplatte_hinten:1
- Passend:93 [Mate]: ISO 7089 3:40 ↔ Kreuz_Halterung:1
- Einfügen:40 [Insert]: ISO 7089 3:40 ↔ Sechskantmutter mit Sicherungselement - Stahl Metrisch Property Class 5 and 10 - Metric M3 x 0.5 Metallisch:20
- Passend:94 [Mate]: ISO 7089 3:41 ↔ Obenplatte_vorne:1
- Passend:95 [Mate]: ISO 7089 3:41 ↔ Obenplatte_vorne:1
- Einfügen:41 [Insert]: ISO 7089 3:41 ↔ BS 4168 : Teil 1 Innensechskantschraube - Metrisch M3 x 8:6
- Passend:96 [Mate]: ISO 7089 3:42 ↔ Obenplatte_vorne:1
- Passend:97 [Mate]: ISO 7089 3:42 ↔ Obenplatte_vorne:1
- Einfügen:42 [Insert]: ISO 7089 3:42 ↔ BS 4168 : Teil 1 Innensechskantschraube - Metrisch M3 x 8:7
- Passend:98 [Mate]: ISO 7089 3:43 ↔ Obenplatte_vorne:1
- Passend:99 [Mate]: ISO 7089 3:43 ↔ Obenplatte_vorne:1
- Einfügen:43 [Insert]: ISO 7089 3:43 ↔ BS 4168 : Teil 1 Innensechskantschraube - Metrisch M3 x 8:8
- Passend:100 [Mate]: ISO 7089 3:44 ↔ Obenplatte_vorne:1
- Passend:101 [Mate]: ISO 7089 3:44 ↔ Obenplatte_vorne:1
- Einfügen:44 [Insert]: ISO 7089 3:44 ↔ BS 4168 : Teil 1 Innensechskantschraube - Metrisch M3 x 8:9
- Passend:102 [Mate]: Obenplatte_hinten:1 ↔ Grundplatte_hinten:1
- Passend:103 [Mate]: Obenplatte_hinten:1 ↔ Grundplatte_hinten:1
- Passend:104 [Mate]: Obenplatte_hinten:1 ↔ Grundplatte_hinten:1
- Passend:105 [Mate]: ISO 7089 3:45 ↔ Obenplatte_hinten:1
- Passend:106 [Mate]: ISO 7089 3:45 ↔ Obenplatte_hinten:1
- Einfügen:45 [Insert]: ISO 7089 3:45 ↔ BS 4168 : Teil 1 Innensechskantschraube - Metrisch M3 x 8:10
- Passend:107 [Mate]: ISO 7089 3:46 ↔ Obenplatte_hinten:1
- Passend:108 [Mate]: ISO 7089 3:46 ↔ Obenplatte_hinten:1
- Einfügen:46 [Insert]: ISO 7089 3:46 ↔ BS 4168 : Teil 1 Innensechskantschraube - Metrisch M3 x 8:11
- Passend:109 [Mate]: ISO 7089 3:47 ↔ Obenplatte_hinten:1
- Passend:110 [Mate]: ISO 7089 3:47 ↔ Obenplatte_hinten:1
- Einfügen:47 [Insert]: ISO 7089 3:47 ↔ BS 4168 : Teil 1 Innensechskantschraube - Metrisch M3 x 8:12
- Passend:111 [Mate]: ISO 7089 3:48 ↔ Obenplatte_hinten:1
- Passend:112 [Mate]: ISO 7089 3:48 ↔ Obenplatte_hinten:1
- Einfügen:48 [Insert]: ISO 7089 3:48 ↔ BS 4168 : Teil 1 Innensechskantschraube - Metrisch M3 x 8:13
- Passend:113 [Mate]: Obenplatte_vorne:1 ↔ Halterung_Differential_3:1
- Passend:114 [Mate]: Obenplatte_hinten:1 ↔ Halterung_Differential_3:1
- Passend:115 [Mate]: Obenplatte_hinten:1 ↔ Halterung_Differential_3:1
- Passend:116 [Mate]: Obenplatte_vorne:1 ↔ Halterung_Differential_3:2
- Passend:117 [Mate]: Obenplatte_hinten:1 ↔ Halterung_Differential_3:2
- Passend:118 [Mate]: Obenplatte_hinten:1 ↔ Halterung_Differential_3:2
- Passend:119 [Mate]: ISO 7089 3:49 ↔ Halterung_Differential_3:2
- Passend:120 [Mate]: ISO 7089 3:49 ↔ Halterung_Differential_3:2
- Einfügen:49 [Insert]: ISO 7089 3:49 ↔ BS 4168 : Teil 1 Innensechskantschraube - Metrisch M3 x 12:1
- Passend:121 [Mate]: ISO 7089 3:50 ↔ Halterung_Differential_3:2
- Passend:122 [Mate]: ISO 7089 3:50 ↔ Obenplatte_hinten:1
- Einfügen:50 [Insert]: ISO 7089 3:50 ↔ Sechskantmutter mit Sicherungselement - Stahl Metrisch Property Class 5 and 10 - Metric M3 x 0.5 Metallisch:21
- Passend:123 [Mate]: ISO 7089 3:51 ↔ Halterung_Differential_3:2
- Passend:124 [Mate]: ISO 7089 3:51 ↔ Halterung_Differential_3:2
- Einfügen:51 [Insert]: ISO 7089 3:51 ↔ BS 4168 : Teil 1 Innensechskantschraube - Metrisch M3 x 12:2
- Passend:125 [Mate]: ISO 7089 3:52 ↔ Halterung_Differential_3:2
- Passend:126 [Mate]: ISO 7089 3:52 ↔ Obenplatte_vorne:1
- Einfügen:52 [Insert]: ISO 7089 3:52 ↔ Sechskantmutter mit Sicherungselement - Stahl Metrisch Property Class 5 and 10 - Metric M3 x 0.5 Metallisch:22
- Passend:127 [Mate]: ISO 7089 3:53 ↔ Halterung_Differential_3:1
- Passend:128 [Mate]: ISO 7089 3:53 ↔ Halterung_Differential_3:1
- Einfügen:53 [Insert]: ISO 7089 3:53 ↔ BS 4168 : Teil 1 Innensechskantschraube - Metrisch M3 x 12:3
- Passend:129 [Mate]: ISO 7089 3:54 ↔ Halterung_Differential_3:1
- Passend:130 [Mate]: ISO 7089 3:54 ↔ Obenplatte_hinten:1
- Einfügen:54 [Insert]: ISO 7089 3:54 ↔ Sechskantmutter mit Sicherungselement - Stahl Metrisch Property Class 5 and 10 - Metric M3 x 0.5 Metallisch:23
- Passend:131 [Mate]: ISO 7089 3:55 ↔ Halterung_Differential_3:1
- Passend:132 [Mate]: ISO 7089 3:55 ↔ Halterung_Differential_3:1
- Einfügen:55 [Insert]: ISO 7089 3:55 ↔ BS 4168 : Teil 1 Innensechskantschraube - Metrisch M3 x 12:4
- Passend:133 [Mate]: ISO 7089 3:56 ↔ Halterung_Differential_3:1
- Passend:134 [Mate]: ISO 7089 3:56 ↔ Obenplatte_vorne:1
- Einfügen:56 [Insert]: ISO 7089 3:56 ↔ Sechskantmutter mit Sicherungselement - Stahl Metrisch Property Class 5 and 10 - Metric M3 x 0.5 Metallisch:24
- Passend:137 [Mate]: Halterung_Differential:2 ↔ Obenplatte_vorne:1
- Passend:140 [Mate]: Halterung_Differential:1 ↔ Obenplatte_hinten:1
- Passend:144 [Mate]: Halterung_Differential:2 ↔ Obenplatte_vorne:1
- Passend:145 [Mate]: Halterung_Differential:2 ↔ Obenplatte_hinten:1
- Passend:146 [Mate]: Halterung_Differential:1 ↔ Obenplatte_hinten:1
- Passend:147 [Mate]: Halterung_Differential:1 ↔ Obenplatte_vorne:1
- Passend:148 [Mate]: Halterung_Differential:1 ↔ Halterung_Differential_2:1
- Passend:149 [Mate]: Halterung_Differential:2 ↔ Halterung_Differential_2:1
- Passend:150 [Mate]: Kugellager:3 ↔ Halterung_Differential_3:2
- Passend:151 [Mate]: Kugellager:3 ↔ Halterung_Differential_3:2
- Passend:152 [Mate]: Halterung_Differential_2:1 ↔ Kugellager:1
- Passend:153 [Mate]: Halterung_Differential_2:1 ↔ Obenplatte_vorne:1
- Passend:154 [Mate]: Halterung_Differential_2:1 ↔ Kugellager:1
- Passend:155 [Mate]: Halterung_Differential:2 ↔ Kugellager:2
- Passend:156 [Mate]: Halterung_Differential:2 ↔ Kugellager:2
- Passend:157 [Mate]: Halterung_Differential:1 ↔ Kugellager:4
- Passend:158 [Mate]: Halterung_Differential:1 ↔ Kugellager:4
- Passend:159 [Mate]: Kugellager:5 ↔ Halterung_Differential_3:1
- Passend:160 [Mate]: Kugellager:5 ↔ Halterung_Differential_3:1
- Passend:161 [Mate]: Halterung_Differential_Mitte:1 ↔ Obenplatte_vorne:1
- Passend:162 [Mate]: Halterung_Differential_Mitte:1 ↔ Obenplatte_vorne:1
- Passend:163 [Mate]: Halterung_Differential_Mitte:1 ↔ Obenplatte_vorne:1
- Passend:164 [Mate]: Halterung_Differential_Mitte:1 ↔ Kugellager_klein:1
- Passend:165 [Mate]: Halterung_Differential_Mitte:1 ↔ Kugellager_klein:1
- Einfügen:57 [Insert] (-4.5 mm): Kugellager_klein:1 ↔ Welle_Kugellager_Mitte:1
- Passend:166 [Mate]: Kegelrad2:1 ↔ Welle_Kugellager_Mitte:1
- Passend:167 [Mate]: Kegelrad2:1 ↔ Welle_Kugellager_Mitte:1
- Einfügen:58 [Insert] (-52 mm): Verbindung_Rocker_Body:2 ↔ Kugellager:5
- Passend:168 [Mate]: Kegelrad2:2 ↔ Verbindung_Rocker_Body:2
- Passend:169 [Mate]: Kegelrad2:2 ↔ Verbindung_Rocker_Body:2
- Winkel:4 [Angle] (0 deg): Kegelrad2:2 ↔ Verbindung_Rocker_Body:2
- Drehung:1 [RelateRotation] (1 ul): Kegelrad2:2 ↔ Kegelrad2:1
- Winkel:5 [Angle] (0 deg): Kegelrad2:1 ↔ Welle_Kugellager_Mitte:1
- Winkel:6 [Angle] (10 deg): Kegelrad2:1 ↔ Obenplatte_vorne:1
- Einfügen:59 [Insert] (-52 mm): Verbindung_Rocker_Body:1 ↔ Kugellager:3
- Passend:170 [Mate]: Kegelrad2:3 ↔ Verbindung_Rocker_Body:1
- Passend:171 [Mate]: Kegelrad2:3 ↔ Verbindung_Rocker_Body:1
- Winkel:7 [Angle] (90 deg): Kegelrad2:3 ↔ Verbindung_Rocker_Body:1
- Drehung:2 [RelateRotation] (1 ul): Kegelrad2:3 ↔ Kegelrad2:1
- Passend:172 [Mate]: ISO 7089 3:57 ↔ Halterung_Differential:2
- Passend:173 [Mate]: ISO 7089 3:57 ↔ Halterung_Differential:2
- Einfügen:60 [Insert]: ISO 7089 3:57 ↔ BS 4168 : Teil 1 Innensechskantschraube - Metrisch M3 x 12:5
- Passend:174 [Mate]: ISO 7089 3:58 ↔ Halterung_Differential:2
- Passend:175 [Mate]: ISO 7089 3:58 ↔ Obenplatte_hinten:1
- Einfügen:61 [Insert]: ISO 7089 3:58 ↔ Sechskantmutter mit Sicherungselement - Stahl Metrisch Property Class 5 and 10 - Metric M3 x 0.5 Metallisch:25
- Passend:176 [Mate]: ISO 7089 3:59 ↔ Halterung_Differential:1
- Passend:177 [Mate]: ISO 7089 3:59 ↔ Halterung_Differential:1
- Einfügen:62 [Insert]: ISO 7089 3:59 ↔ BS 4168 : Teil 1 Innensechskantschraube - Metrisch M3 x 12:6
- Passend:178 [Mate]: ISO 7089 3:60 ↔ Halterung_Differential:1
- Passend:179 [Mate]: ISO 7089 3:60 ↔ Obenplatte_hinten:1
- Einfügen:63 [Insert]: ISO 7089 3:60 ↔ Sechskantmutter mit Sicherungselement - Stahl Metrisch Property Class 5 and 10 - Metric M3 x 0.5 Metallisch:26
- Passend:180 [Mate]: ISO 7089 3:61 ↔ Halterung_Differential_2:1
- Passend:181 [Mate]: ISO 7089 3:61 ↔ Halterung_Differential_2:1
- Einfügen:64 [Insert]: ISO 7089 3:61 ↔ BS 4168 : Teil 1 Innensechskantschraube - Metrisch M3 x 16:1
- Passend:182 [Mate]: ISO 7089 3:62 ↔ Halterung_Differential_2:1
- Passend:183 [Mate]: ISO 7089 3:62 ↔ Obenplatte_vorne:1
- Einfügen:65 [Insert]: ISO 7089 3:62 ↔ Sechskantmutter mit Sicherungselement - Stahl Metrisch Property Class 5 and 10 - Metric M3 x 0.5 Metallisch:27
- Passend:184 [Mate]: ISO 7089 3:63 ↔ Halterung_Differential_Mitte:1
- Passend:185 [Mate]: ISO 7089 3:63 ↔ Halterung_Differential_Mitte:1
- Einfügen:66 [Insert]: ISO 7089 3:63 ↔ BS 4168 : Teil 1 Innensechskantschraube - Metrisch M3 x 12:7
- Passend:186 [Mate]: ISO 7089 3:64 ↔ Halterung_Differential_Mitte:1
- Passend:187 [Mate]: ISO 7089 3:64 ↔ Obenplatte_vorne:1
- Einfügen:67 [Insert]: ISO 7089 3:64 ↔ Sechskantmutter mit Sicherungselement - Stahl Metrisch Property Class 5 and 10 - Metric M3 x 0.5 Metallisch:28
- Passend:188 [Mate]: ISO 7089 3:65 ↔ Halterung_Differential_Mitte:1
- Passend:189 [Mate]: ISO 7089 3:65 ↔ Halterung_Differential_Mitte:1
- Einfügen:68 [Insert]: ISO 7089 3:65 ↔ BS 4168 : Teil 1 Innensechskantschraube - Metrisch M3 x 12:8
- Passend:190 [Mate]: ISO 7089 3:66 ↔ Halterung_Differential_Mitte:1
- Passend:191 [Mate]: ISO 7089 3:66 ↔ Obenplatte_vorne:1
- Einfügen:69 [Insert]: ISO 7089 3:66 ↔ Sechskantmutter mit Sicherungselement - Stahl Metrisch Property Class 5 and 10 - Metric M3 x 0.5 Metallisch:29
- Passend:192 [Mate]: ISO 7089 3:67 ↔ Halterung_Differential_2:1
- Passend:193 [Mate]: ISO 7089 3:67 ↔ Halterung_Differential_2:1
- Einfügen:70 [Insert]: ISO 7089 3:67 ↔ BS 4168 : Teil 1 Innensechskantschraube - Metrisch M3 x 16:2
- Passend:194 [Mate]: ISO 7089 3:68 ↔ Halterung_Differential_2:1
- Passend:195 [Mate]: ISO 7089 3:68 ↔ Obenplatte_vorne:1
- Einfügen:71 [Insert]: ISO 7089 3:68 ↔ Sechskantmutter mit Sicherungselement - Stahl Metrisch Property Class 5 and 10 - Metric M3 x 0.5 Metallisch:30
- Passend:196 [Mate]: Fahrwerk_rocker_hinten:1 ↔ Verbindung_Rocker_Body:2
- Passend:197 [Mate]: Fahrwerk_rocker_hinten:1 ↔ Verbindung_Rocker_Body:2
- Winkel:8 [Angle] (0 deg): Fahrwerk_rocker_hinten:1 ↔ Verbindung_Rocker_Body:2
- Passend:198 [Mate]: Fahrwerk_rocker_hinten:2 ↔ Verbindung_Rocker_Body:1
- Passend:199 [Mate]: Fahrwerk_rocker_hinten:2 ↔ Verbindung_Rocker_Body:1
- Winkel:9 [Angle] (0 deg): Fahrwerk_rocker_hinten:2 ↔ Verbindung_Rocker_Body:1
- Passend:200 [Mate]: Fahrwerk_rocker_hinten:1 ↔ Kugellager:6
- Passend:201 [Mate]: Fahrwerk_rocker_hinten:1 ↔ Kugellager:6
- Passend:202 [Mate]: Fahrwerk_rocker_hinten:1 ↔ Kugellager:7
- Passend:203 [Mate]: Fahrwerk_rocker_hinten:1 ↔ Kugellager:7
- Einfügen:72 [Insert] (-22 mm): Kugellager:6 ↔ Boogie_Stange:1
- Passend:204 [Mate]: Boogie_Stange:1 ↔ Fahrwerk_bogie:1
- Passend:205 [Mate]: Boogie_Stange:1 ↔ Fahrwerk_bogie:1
- Winkel:10 [Angle] (0 deg): Boogie_Stange:1 ↔ Fahrwerk_bogie:1
